# Autodesk Inventor assembly: podwojne koło zebate_MIR
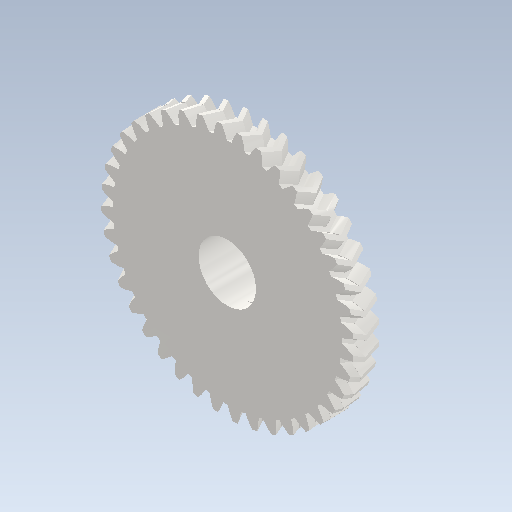
[picture p0: Inventor's stored thumbnail of the model, 512x512]
Saved by Autodesk Inventor 2021 (Build 250183000, 183)
## iProperties
Created: 2021-06-27
Part Number: podwojne koło zebate_MIR
Document SubType Name: Assembly
Designer: Łukasz
Author: Łukasz
## Documents named in this file (3)
- E:\GITHUB_Czołg\Szybki-Czolg-antyRadziecki\koła zębate\Design Accelerator\podwojne koło zebate_MIR.iam
- E:\GITHUB_Czołg\Szybki-Czolg-antyRadziecki\koła zębate\Design Accelerator\inny set zebow\Design Accelerator\Spur Gear21_MIR.ipt
- E:\GITHUB_Czołg\Szybki-Czolg-antyRadziecki\koła zębate\Design Accelerator\inny set zebow\Design Accelerator\Spur Gear11_MIR.ipt
## Components (2 placed, 2 different names)
1. Spur Gear21_MIR:1 — Rigid:1
2. Spur Gear11_MIR:1 — Rigid:1
## Relationships (1: WeldJoint 1)
- Rigid:1 [WeldJoint]: Spur Gear21_MIR:1 ↔ Spur Gear11_MIR:1
